# Autodesk Inventor assembly: Ролик натяжителя
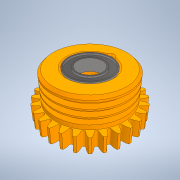
[picture p0: Inventor's stored thumbnail of the model, 180x180]
Saved by Autodesk Inventor 2021.1 (Build 251245010, 245A)
## iProperties
Created: 2026-05-05
Part Number: Ролик натяжителя
Document SubType Name: Assembly
Designer: Андрей Тарасов
Author: Андрей Тарасов
## Documents named in this file (3)
- G:\04. Inventor\024. EDM 3.0\Ролик натяжителя.iam
- G:\04. Inventor\024. EDM 3.0\Подшипник 8х14х4.ipt
- G:\04. Inventor\024. EDM 3.0\Ролик с шестерней.ipt
## Components (3 placed, 2 different names)
1. Подшипник 8х14х4:1 — Совмещение:1, Заподлицо:1
2. Подшипник 8х14х4:2 — Совмещение:2, Заподлицо:2
3. Ролик с шестерней:1 — Совмещение:1, Заподлицо:1, Совмещение:2, Заподлицо:2
## Relationships (4: Mate 2, Flush 2)
- Совмещение:1 [Mate]: Подшипник 8х14х4:1 ↔ Ролик с шестерней:1
- Заподлицо:1 [Flush]: Подшипник 8х14х4:1 ↔ Ролик с шестерней:1
- Совмещение:2 [Mate]: Подшипник 8х14х4:2 ↔ Ролик с шестерней:1
- Заподлицо:2 [Flush]: Подшипник 8х14х4:2 ↔ Ролик с шестерней:1
